# Autodesk Inventor assembly: ENCODER ASSY
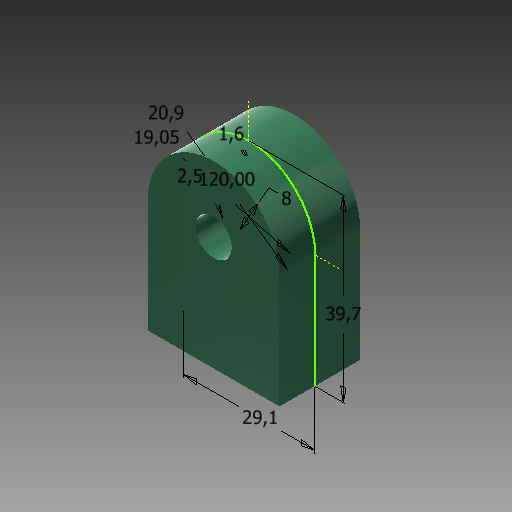
[picture p0: Inventor's stored thumbnail of the model, 512x512]
Saved by Autodesk Inventor 2018.3 (Build 223284000, 284)
## iProperties
Created: 2012-07-24
Part Number: ENCODER ASSY
Material: Generisch
Description: STEP AP214
Document SubType Name: Assembly
Designer: JochenAlt
Sending System: SolidWorks 2011
Preprocessor: SwSTEP 2.0
Title: ENCODER ASSY.STEP
Revision Number: ANY
## Documents named in this file (4)
- D:\Projects\Ondine\CAD\Encoder\Avago Encoder.iam
- D:\Projects\Ondine\CAD\Encoder\HEDS-9040.ipt
- D:\Projects\Ondine\CAD\Encoder\HEDM-512.ipt
- D:\Projects\Ondine\CAD\Encoder\EncoderEnclosure.ipt
## Components (3 placed, 3 different names)
1. HEDS-9040_1
2. HEDM-512_2
3. EncoderEnclosure:1 — Fluchtend:1, Fluchtend:2
## Relationships (2: Flush 2)
- Fluchtend:1 [Flush]: EncoderEnclosure:1
- Fluchtend:2 [Flush]: EncoderEnclosure:1
